# Autodesk Inventor assembly: assembly
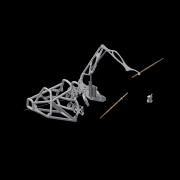
[picture p0: Inventor's stored thumbnail of the model, 180x180]
Saved by Autodesk Inventor 2020 (Build 240168000, 168)
## iProperties
Created: 2020-03-24
Part Number: assembly
Document SubType Name: Assembly
Designer: valer
Author: valer
## Documents named in this file (24)
- C:\Users\valer\Desktop\drummingrobot\src\Robot.iam
- C:\Users\valer\Desktop\drummingrobot\src\Chest.ipt
- C:\Users\valer\Desktop\drummingrobot\src\HeadScaled.ipt
- C:\Users\valer\Desktop\drummingrobot\src\UpperArm.ipt
- C:\Users\valer\Desktop\drummingrobot\src\UpperArmBracket.ipt
- C:\Users\valer\Desktop\drummingrobot\src\external\ShoulderConnectingRod.ipt
- C:\Users\valer\Desktop\drummingrobot\src\Forearm.ipt
- C:\Users\valer\Desktop\drummingrobot\src\external\Drumstick.ipt
- C:\Users\valer\Desktop\drummingrobot\src\external\ForearmShaftCollar.ipt
- C:\Users\valer\Desktop\drummingrobot\src\external\RodEndFixed.ipt
- C:\Users\valer\Desktop\drummingrobot\src\ShoulderBracket.ipt
- C:\Users\valer\Desktop\drummingrobot\src\ChestShoulderBracket.ipt
- C:\Users\valer\Desktop\drummingrobot\src\ChestShoulderBracketMirror.ipt
- C:\Users\valer\Desktop\drummingrobot\src\external\PullSolenoid.ipt
- C:\Users\valer\Desktop\drummingrobot\src\external\PushSolenoid.ipt
- C:\Users\valer\Desktop\drummingrobot\src\external\UpperArmActuatorBody.ipt
- C:\Users\valer\Desktop\drummingrobot\src\external\UpperArmActuatorShaft.ipt
- C:\Users\valer\Desktop\drummingrobot\src\external\ForearmActuatorBody.ipt
- C:\Users\valer\Desktop\drummingrobot\src\external\ForearmActuatorShaft.ipt
- C:\Users\valer\Desktop\drummingrobot\src\external\Drums.ipt
- C:\Users\valer\Desktop\drummingrobot\src\ForearmActuatorConnector.ipt
- C:\Users\valer\Desktop\drummingrobot\src\UpperArmBracketMirror.ipt
- C:\Users\valer\Desktop\drummingrobot\src\UpperArmActuatorBracket.ipt
- C:\Users\valer\Desktop\drummingrobot\src\UpperArmActuatorBracketMirror.ipt
## Components (53 placed, 22 different names)
1. Chest:1 — Angle:6, Mate:117, Mate:118, Mate:119, Mate:120, Mate:121, Mate:122, Mate:130, Mate:131, Mate:132, Mate:133, Mate:134, Mate:157
2. HeadScaled:1 — Angle:6
3. ChestConnectingRod:1 — Mate:88, Mate:89, Mate:105
4. ChestConnectingRod:2 — Mate:86, Mate:87, Mate:104
5. ChestConnectingRod:3 — Mate:84, Mate:85, Mate:98
6. ChestConnectingRod:4 — Mate:82, Mate:83, Mate:97
7. Drumstick:1 — Mate:79, Flush:3
8. ShaftCollar1/2:1 — Mate:79, Flush:3, Mate:236, Flush:18
9. RodEnd1/4-1/4-1:1 — Mate:82, Mate:115
10. RodEnd1/4-1/4-1:2 — Mate:83, Mate:97, Mate:123, Mate:125
11. RodEnd1/4-1/4-1:3 — Mate:84, Mate:114
12. RodEnd1/4-1/4-1:4 — Mate:85, Mate:98, Mate:124, Mate:142
13. RodEnd1/4-1/4-1:5 — Mate:86, Mate:110
14. RodEnd1/4-1/4-1:6 — Mate:87, Mate:104, Mate:126, Mate:129
15. RodEnd1/4-1/4-1:7 — Mate:88, Mate:109
16. RodEnd1/4-1/4-1:8 — Mate:89, Mate:105, Mate:127, Mate:128
17. ShoulderBracket:2 — Mate:109, Mate:110, Flush:6, Flush:9, Flush:14
18. ShoulderBracket:3 — Flush:6, Mate:114, Mate:115, Flush:8, Flush:14
19. ChestShoulderBracket:1 — Mate:120, Mate:121, Mate:122, Mate:123, Mate:124, Flush:8, Mate:125, Mate:142
20. ChestShoulderBracketMirror:1 — Mate:117, Mate:118, Mate:119, Mate:126, Mate:127, Flush:9, Mate:128, Mate:129
21. ChestShoulderBracket:2 — Mate:130, Mate:131, Mate:157, Mate:160, Mate:162, Mate:213, Mate:214
22. ShoulderBracket:4 — Mate:144, Mate:145, Mate:147, Flush:15
23. ShoulderBracket:5 — Mate:159, Mate:209, Mate:211, Mate:212, Flush:15
24. ChestShoulderBracketMirror:2 — Mate:132, Mate:133, Mate:134, Mate:141, Mate:146, Mate:148, Mate:149
25. ChestConnectingRod:5
26. ChestConnectingRod:6
27. RodEnd1/4-1/4-1:9 — Mate:144, Mate:145
28. RodEnd1/4-1/4-1:10 — Mate:148, Mate:149
29. RodEnd1/4-1/4-1:11 — Mate:147
30. RodEnd1/4-1/4-1:12 — Mate:141, Mate:146
31. ChestConnectingRod:7
32. ChestConnectingRod:8
33. RodEnd1/4-1/4-1:13 — Mate:211, Mate:212
34. RodEnd1/4-1/4-1:14 — Mate:162, Mate:214
35. RodEnd1/4-1/4-1:15 — Mate:159, Mate:209
36. RodEnd1/4-1/4-1:16 — Mate:160, Mate:213
37. Drumstick:2 — Mate:181
38. ShaftCollar1/2:2 — Mate:181
39. PullSolenoid:1
40. PushSolenoid:1
41. FA-35-S-12-1:1 — Mate:182, Mate:183, Mate:257
42. Forearm:1 — Flush:17, Mate:227, Mate:236, Flush:18, Mate:239, Mate:244
43. FA-35-S-12-1:2 — Mate:182, Mate:183, Mate:238, Flush:20
44. ForearmActuatorBody:1 — Mate:231, Mate:232, Mate:234, Flush:19
45. Drums:1 — Flush:13
46. ForearmActuatorShaft:3 — Flush:17, Mate:231, Mate:232, Mate:241, Mate:243, Angle:10, Mate:246
47. UpperArm:3 — Mate:227, Mate:234, Mate:238, Flush:19, Flush:20, Mate:247, Mate:248, Mate:249, Mate:250
48. ForearmActuatorConnector:1 — Mate:239, Mate:241, Mate:245, Angle:10, Mate:246
49. ForearmActuatorConnector:2 — Mate:243, Mate:244, Mate:245
50. UpperArmBracket:5 — Mate:249, Mate:250, Mate:254, Mate:255, Mate:256, Flush:21
51. UpperArmBracketMirror:1 — Mate:247, Mate:248, Mate:251, Mate:252, Mate:253, Flush:21
52. UpperArmActuatorBracket:1 — Mate:254, Mate:255, Mate:256
53. UpperArmActuatorBracketMirror:1 — Mate:251, Mate:252, Mate:253, Mate:257
## Relationships (106: Mate 90, Flush 14, Angle 2)
- Angle:6 (0 deg): Chest:1 ↔ HeadScaled:1
- Mate:79: Drumstick:1 ↔ ShaftCollar1/2:1
- Flush:3 (304.8 mm): Drumstick:1 ↔ ShaftCollar1/2:1
- Mate:82: ChestConnectingRod:4 ↔ RodEnd1/4-1/4-1:1
- Mate:83: ChestConnectingRod:4 ↔ RodEnd1/4-1/4-1:2
- Mate:84: ChestConnectingRod:3 ↔ RodEnd1/4-1/4-1:3
- Mate:85: ChestConnectingRod:3 ↔ RodEnd1/4-1/4-1:4
- Mate:86: ChestConnectingRod:2 ↔ RodEnd1/4-1/4-1:5
- Mate:87: ChestConnectingRod:2 ↔ RodEnd1/4-1/4-1:6
- Mate:88: ChestConnectingRod:1 ↔ RodEnd1/4-1/4-1:7
- Mate:89: ChestConnectingRod:1 ↔ RodEnd1/4-1/4-1:8
- Mate:97 (-25.4 mm): ChestConnectingRod:4 ↔ RodEnd1/4-1/4-1:2
- Mate:98 (-25.4 mm): ChestConnectingRod:3 ↔ RodEnd1/4-1/4-1:4
- Mate:104 (-25.4 mm): ChestConnectingRod:2 ↔ RodEnd1/4-1/4-1:6
- Mate:105 (-25.4 mm): ChestConnectingRod:1 ↔ RodEnd1/4-1/4-1:8
- Mate:109: RodEnd1/4-1/4-1:7 ↔ ShoulderBracket:2
- Mate:110: RodEnd1/4-1/4-1:5 ↔ ShoulderBracket:2
- Flush:6: ShoulderBracket:2 ↔ ShoulderBracket:3
- Mate:114: RodEnd1/4-1/4-1:3 ↔ ShoulderBracket:3
- Mate:115: RodEnd1/4-1/4-1:1 ↔ ShoulderBracket:3
- Mate:117: Chest:1 ↔ ChestShoulderBracketMirror:1
- Mate:118: Chest:1 ↔ ChestShoulderBracketMirror:1
- Mate:119: Chest:1 ↔ ChestShoulderBracketMirror:1
- Mate:120: Chest:1 ↔ ChestShoulderBracket:1
- Mate:121: Chest:1 ↔ ChestShoulderBracket:1
- Mate:122: Chest:1 ↔ ChestShoulderBracket:1
- Mate:123: RodEnd1/4-1/4-1:2 ↔ ChestShoulderBracket:1
- Mate:124: RodEnd1/4-1/4-1:4 ↔ ChestShoulderBracket:1
- Flush:8: ShoulderBracket:3 ↔ ChestShoulderBracket:1
- Mate:125: RodEnd1/4-1/4-1:2 ↔ ChestShoulderBracket:1
- Mate:126: RodEnd1/4-1/4-1:6 ↔ ChestShoulderBracketMirror:1
- Mate:127: RodEnd1/4-1/4-1:8 ↔ ChestShoulderBracketMirror:1
- Flush:9: ShoulderBracket:2 ↔ ChestShoulderBracketMirror:1
- Mate:128: RodEnd1/4-1/4-1:8 ↔ ChestShoulderBracketMirror:1
- Mate:129: RodEnd1/4-1/4-1:6 ↔ ChestShoulderBracketMirror:1
- Mate:130: Chest:1 ↔ ChestShoulderBracket:2
- Mate:131: Chest:1 ↔ ChestShoulderBracket:2
- [Flush]: ShoulderBracket:4 ↔ ShoulderBracket:5
- Mate:132: Chest:1 ↔ ChestShoulderBracketMirror:2
- Mate:133: Chest:1 ↔ ChestShoulderBracketMirror:2
- Mate:134: Chest:1 ↔ ChestShoulderBracketMirror:2
- [Mate]: ChestConnectingRod:6 ↔ RodEnd1/4-1/4-1:9
- [Mate]: ChestConnectingRod:6 ↔ RodEnd1/4-1/4-1:10
- [Mate]: ChestConnectingRod:5 ↔ RodEnd1/4-1/4-1:11
- [Mate]: ChestConnectingRod:5 ↔ RodEnd1/4-1/4-1:12
- [Mate] (-25.4 mm): ChestConnectingRod:6 ↔ RodEnd1/4-1/4-1:10
- [Mate] (-25.4 mm): ChestConnectingRod:5 ↔ RodEnd1/4-1/4-1:12
- Mate:141: ChestShoulderBracketMirror:2 ↔ RodEnd1/4-1/4-1:12
- Mate:142: RodEnd1/4-1/4-1:4 ↔ ChestShoulderBracket:1
- Mate:144: ShoulderBracket:4 ↔ RodEnd1/4-1/4-1:9
- Mate:145: ShoulderBracket:4 ↔ RodEnd1/4-1/4-1:9
- Mate:146: ChestShoulderBracketMirror:2 ↔ RodEnd1/4-1/4-1:12
- Mate:147: ShoulderBracket:4 ↔ RodEnd1/4-1/4-1:11
- Mate:148: ChestShoulderBracketMirror:2 ↔ RodEnd1/4-1/4-1:10
- Mate:149: ChestShoulderBracketMirror:2 ↔ RodEnd1/4-1/4-1:10
- [Mate]: ChestConnectingRod:8 ↔ RodEnd1/4-1/4-1:13
- [Mate]: ChestConnectingRod:8 ↔ RodEnd1/4-1/4-1:14
- [Mate]: ChestConnectingRod:7 ↔ RodEnd1/4-1/4-1:15
- [Mate]: ChestConnectingRod:7 ↔ RodEnd1/4-1/4-1:16
- [Mate] (-25.4 mm): ChestConnectingRod:8 ↔ RodEnd1/4-1/4-1:14
- [Mate] (-25.4 mm): ChestConnectingRod:7 ↔ RodEnd1/4-1/4-1:16
- Mate:157: Chest:1 ↔ ChestShoulderBracket:2
- Mate:159: ShoulderBracket:5 ↔ RodEnd1/4-1/4-1:15
- Mate:160: ChestShoulderBracket:2 ↔ RodEnd1/4-1/4-1:16
- Mate:162: ChestShoulderBracket:2 ↔ RodEnd1/4-1/4-1:14
- [Flush] (304.8 mm): Drumstick:2 ↔ ShaftCollar1/2:2
- Mate:181: Drumstick:2 ↔ ShaftCollar1/2:2
- Mate:182: FA-35-S-12-1:1 ↔ FA-35-S-12-1:2
- Mate:183: FA-35-S-12-1:1 ↔ FA-35-S-12-1:2
- Flush:13 (508 mm): Drums:1
- Flush:14: ShoulderBracket:2 ↔ ShoulderBracket:3
- Mate:209: ShoulderBracket:5 ↔ RodEnd1/4-1/4-1:15
- Mate:211: ShoulderBracket:5 ↔ RodEnd1/4-1/4-1:13
- Mate:212: ShoulderBracket:5 ↔ RodEnd1/4-1/4-1:13
- Mate:213: ChestShoulderBracket:2 ↔ RodEnd1/4-1/4-1:16
- Mate:214: ChestShoulderBracket:2 ↔ RodEnd1/4-1/4-1:14
- Flush:15: ShoulderBracket:4 ↔ ShoulderBracket:5
- Flush:17: Forearm:1 ↔ ForearmActuatorShaft:3
- Mate:227: Forearm:1 ↔ UpperArm:3
- Mate:231: ForearmActuatorBody:1 ↔ ForearmActuatorShaft:3
- Mate:232: ForearmActuatorBody:1 ↔ ForearmActuatorShaft:3
- Mate:234: ForearmActuatorBody:1 ↔ UpperArm:3
- Mate:236: ShaftCollar1/2:1 ↔ Forearm:1
- Flush:18 (12.7 mm): ShaftCollar1/2:1 ↔ Forearm:1
- Mate:238: FA-35-S-12-1:2 ↔ UpperArm:3
- Flush:19: ForearmActuatorBody:1 ↔ UpperArm:3
- Flush:20: FA-35-S-12-1:2 ↔ UpperArm:3
- Mate:239: Forearm:1 ↔ ForearmActuatorConnector:1
- Mate:241: ForearmActuatorShaft:3 ↔ ForearmActuatorConnector:1
- Mate:243: ForearmActuatorShaft:3 ↔ ForearmActuatorConnector:2
- Mate:244: Forearm:1 ↔ ForearmActuatorConnector:2
- Mate:245: ForearmActuatorConnector:1 ↔ ForearmActuatorConnector:2
- Angle:10 (-180 deg): ForearmActuatorShaft:3 ↔ ForearmActuatorConnector:1
- Mate:246: ForearmActuatorShaft:3 ↔ ForearmActuatorConnector:1
- Mate:247: UpperArm:3 ↔ UpperArmBracketMirror:1
- Mate:248: UpperArm:3 ↔ UpperArmBracketMirror:1
- Mate:249: UpperArm:3 ↔ UpperArmBracket:5
- Mate:250: UpperArm:3 ↔ UpperArmBracket:5
- Mate:251: UpperArmBracketMirror:1 ↔ UpperArmActuatorBracketMirror:1
- Mate:252: UpperArmBracketMirror:1 ↔ UpperArmActuatorBracketMirror:1
- Mate:253: UpperArmBracketMirror:1 ↔ UpperArmActuatorBracketMirror:1
- Mate:254: UpperArmBracket:5 ↔ UpperArmActuatorBracket:1
- Mate:255: UpperArmBracket:5 ↔ UpperArmActuatorBracket:1
- Mate:256: UpperArmBracket:5 ↔ UpperArmActuatorBracket:1
- Flush:21: UpperArmBracket:5 ↔ UpperArmBracketMirror:1
- Mate:257: FA-35-S-12-1:1 ↔ UpperArmActuatorBracketMirror:1
## Named parameters: d236_d209 = 0 mm, d244_d149 = 0 mm, d245_d150 = 0 mm, d246_d151 = 0 mm, d247_d152 = 0 mm, d248_d197 = -25.4 mm, d249_d198 = -25.4 mm, d259_d145 = 0 mm, d260_d146 = 0 mm, d261_d147 = 0 mm, d262_d148 = 0 mm, d263_d190 = -25.4 mm, d264_d191 = -25.4 mm, d276_d142 = 304.8 mm
